# Autodesk Inventor assembly: Arm_MiniLink_Shim_i_8
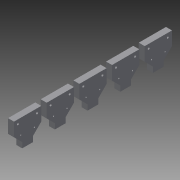
[picture p0: Inventor's stored thumbnail of the model, 180x180]
Saved by Autodesk Inventor 2013 (Build 170138000, 138)
## iProperties
Created: 2014-05-17
Part Number: Arm_MiniLink_Shim_i_8
Document SubType Name: Assembly
Designer: andou
Author: andou
## Documents named in this file (2)
- C:\Users\andou\Documents\Inventor\RoboticsProject\project_4\Robot\Arm\Arm_MiniLink_Shim_5.iam
- C:\Users\andou\Documents\Inventor\RoboticsProject\project_4\Robot\Arm\Arm_MiniLink_Shim.ipt
## Components (5 placed, 1 different names)
1. Arm_MiniLink_Shim:1
2. Arm_MiniLink_Shim:2
3. Arm_MiniLink_Shim:3
4. Arm_MiniLink_Shim:4
5. Arm_MiniLink_Shim:5
## Component patterns: (5 elements, first: Arm_MiniLink_Shim:1)
